# Autodesk Inventor assembly: Bracket and Screws
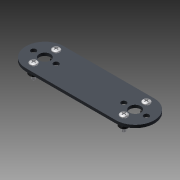
[picture p0: Inventor's stored thumbnail of the model, 180x180]
Saved by Autodesk Inventor 2015 (Build 190159000, 159)
## iProperties
Created: 2014-10-13
Part Number: Bracket and Screws
Document SubType Name: Assembly
Designer: lethcoec
Author: lethcoec
## Documents named in this file (3)
- \\st-svr\studenthdrives$\18\LethcoeC\IED - Lethcoe\FTC Inventor\FTC Parts\Subassemblies\Bracket and Screws.iam
- \\st-svr\studenthdrives$\18\LethcoeC\IED - Lethcoe\FTC Inventor\FTC Parts\Subassemblies\Screw and nut.iam
- \\st-svr\studenthdrives$\18\LethcoeC\IED - Lethcoe\FTC Inventor\Imported Components\BracketFlat\BracketFlat.ipt
## Components (5 placed, 2 different names)
1. Screw and nut:1 [sub-assembly] — Mate:1, Mate:2
2. Screw and nut:2 [sub-assembly] — Mate:5, Mate:6
3. Screw and nut:3 [sub-assembly] — Mate:7, Mate:8
4. Screw and nut:4 [sub-assembly] — Mate:3, Mate:4
5. BracketFlat:1 — Mate:1, Mate:2, Mate:3, Mate:4, Mate:5, Mate:6, Mate:7, Mate:8
## Relationships (8: Mate 8)
- Mate:1: Screw and nut:1 ↔ BracketFlat:1
- Mate:2: Screw and nut:1 ↔ BracketFlat:1
- Mate:3: Screw and nut:4 ↔ BracketFlat:1
- Mate:4: Screw and nut:4 ↔ BracketFlat:1
- Mate:5: Screw and nut:2 ↔ BracketFlat:1
- Mate:6: Screw and nut:2 ↔ BracketFlat:1
- Mate:7: Screw and nut:3 ↔ BracketFlat:1
- Mate:8: Screw and nut:3 ↔ BracketFlat:1
